# Autodesk Inventor assembly: ChupitaTry2
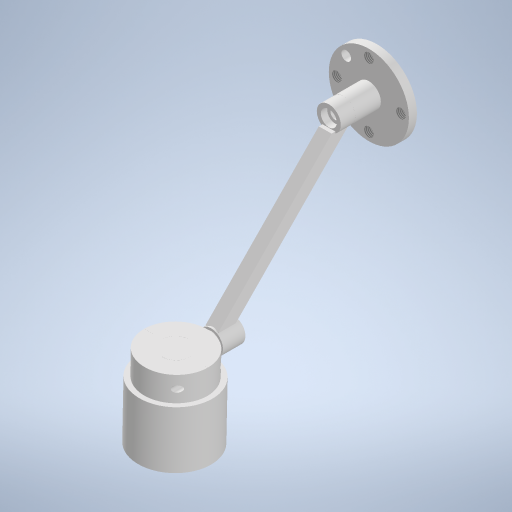
[picture p0: Inventor's stored thumbnail of the model, 512x512]
Saved by Autodesk Inventor 2023 (Build 270158000, 158)
## iProperties
Created: 2022-11-05
Part Number: ChupitaTry2
Document SubType Name: Assembly
Designer: ivanm
Author: ivanm
## Documents named in this file (6)
- C:\Users\ivanm\OneDrive\Robotica\Proyecto-Rob\Piezas\PortaHerramienta\ChupitaTry2.iam
- C:\Users\ivanm\OneDrive\Robotica\Proyecto-Rob\Piezas\PortaHerramienta\Base.ipt
- C:\Users\ivanm\OneDrive\Robotica\Proyecto-Rob\Piezas\PortaHerramienta\Conector.ipt
- C:\Users\ivanm\OneDrive\Robotica\Proyecto-Rob\Piezas\PortaHerramienta\Parte1.ipt
- C:\Users\ivanm\OneDrive\Robotica\Proyecto-Rob\Piezas\PortaHerramienta\Parte2.ipt
- C:\Users\ivanm\OneDrive\Robotica\Proyecto-Rob\Piezas\PortaHerramienta\ModeloSimplificadoVentosa.ipt
## Components (5 placed, 5 different names)
1. Base:1 — Mate:1, Insert:1
2. Conector:1 — Mate:1, Mate:2, Insert:1, Insert:2
3. Parte1:1 — Mate:2, Mate:3, Insert:2, Insert:3, Insert:4, Flush:1, Insert:5
4. Parte2:1 — Mate:3, Insert:3, Insert:4
5. ModeloSimplificadoVentosa:1 — Flush:1, Insert:5
## Relationships (9: Insert 5, Mate 3, Flush 1)
- Mate:1: Base:1 ↔ Conector:1
- Mate:2: Conector:1 ↔ Parte1:1
- Mate:3: Parte1:1 ↔ Parte2:1
- Insert:1: Base:1 ↔ Conector:1
- Insert:2: Conector:1 ↔ Parte1:1
- Insert:3: Parte1:1 ↔ Parte2:1
- Insert:4: Parte1:1 ↔ Parte2:1
- Flush:1: Parte1:1 ↔ ModeloSimplificadoVentosa:1
- Insert:5: Parte1:1 ↔ ModeloSimplificadoVentosa:1
